# Autodesk Inventor assembly: Assembly1
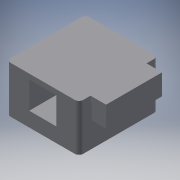
[picture p0: Inventor's stored thumbnail of the model, 180x180]
Saved by Autodesk Inventor 2017 (Build 210142000, 142)
## iProperties
Created: 2018-02-12
Part Number: Assembly1
Document SubType Name: Assembly
Designer: Tripl_000
Author: Tripl_000
## Documents named in this file (3)
- C:\Users\Tripl_000\Desktop\Spira\3D Models\2017\Optical Density Sensor Enclosure\Enclosure\Design 6\Assembly1.iam
- C:\Users\Tripl_000\Desktop\Spira\3D Models\2017\Optical Density Sensor Enclosure\Enclosure\Design 6\Enclosure_Bottom V1D6.ipt
- C:\Users\Tripl_000\Desktop\Spira\3D Models\2017\Optical Density Sensor Enclosure\Enclosure\Design 6\Enclosure_Top V1D6.ipt
## Components (2 placed, 2 different names)
1. Enclosure_Bottom V1D6:1 — Mate:1, Mate:2
2. Enclosure_Top V1D6:1 — Mate:1, Mate:2
## Relationships (2: Mate 2)
- Mate:1: Enclosure_Bottom V1D6:1 ↔ Enclosure_Top V1D6:1
- Mate:2: Enclosure_Bottom V1D6:1 ↔ Enclosure_Top V1D6:1
